# Autodesk Inventor assembly: Tracker V3
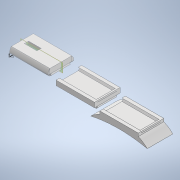
[picture p0: Inventor's stored thumbnail of the model, 180x180]
Saved by Autodesk Inventor 2020 (Build 240168000, 168)
## iProperties
Created: 2019-07-16
Part Number: Tracker V3
Document SubType Name: Assembly
Designer: tyrre
Author: tyrre
## Documents named in this file (4)
- C:\Users\tyrre\OneDrive\Desktop\University - Ryan\Work\Work - 2019\Inventor Files\Tracker V3\Tracker V3.iam
- C:\Users\tyrre\OneDrive\Desktop\University - Ryan\Work\Work - 2019\Inventor Files\Tracker V3\Enclosure-Bottom.ipt
- C:\Users\tyrre\OneDrive\Desktop\University - Ryan\Work\Work - 2019\Inventor Files\Tracker V3\Enclosure-Top.ipt
- C:\Users\tyrre\OneDrive\Desktop\University - Ryan\Work\Work - 2019\Inventor Files\Tracker V3\Enclosure-Base.ipt
## Components (3 placed, 3 different names)
1. Enclosure-Bottom:1 — Mate:1, Mate:2, Flush:1, Mate:3, Mate:4, Flush:2, Mate:5
2. Enclosure-Top:1 — Mate:1, Mate:2, Flush:1
3. Enclosure-Base:1 — Mate:3, Mate:4, Flush:2, Mate:5
## Relationships (7: Mate 5, Flush 2)
- Mate:1: Enclosure-Bottom:1 ↔ Enclosure-Top:1
- Mate:2: Enclosure-Bottom:1 ↔ Enclosure-Top:1
- Flush:1: Enclosure-Bottom:1 ↔ Enclosure-Top:1
- Mate:3: Enclosure-Bottom:1 ↔ Enclosure-Base:1
- Mate:4: Enclosure-Bottom:1 ↔ Enclosure-Base:1
- Flush:2: Enclosure-Bottom:1 ↔ Enclosure-Base:1
- Mate:5: Enclosure-Bottom:1 ↔ Enclosure-Base:1
